# Autodesk Inventor assembly: Ensamblaje2
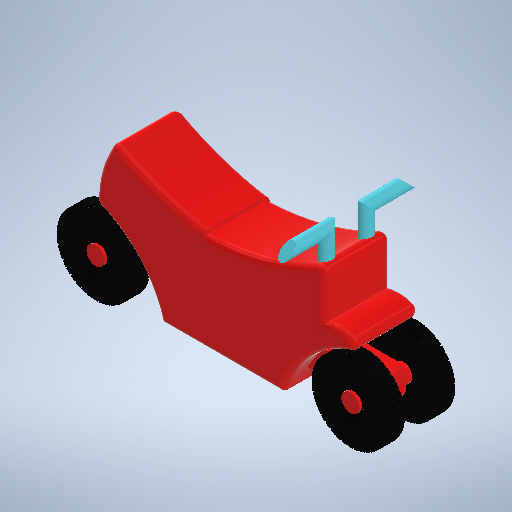
[picture p0: Inventor's stored thumbnail of the model, 512x512]
Saved by Autodesk Inventor 2025.2 (Build 292293000, 293)
## iProperties
Created: 2024-11-29
Part Number: Ensamblaje2
Document SubType Name: Assembly
Designer: usuario
Author: usuario
## Documents named in this file (3)
- C:\Users\usuario\Desktop\APM\ModeladosAPM\Ensamblaje2.iam
- C:\Users\usuario\Desktop\APM\ModeladosAPM\Ensamblajemotocorta.iam
- C:\Users\usuario\Desktop\APM\ModeladosAPM\rueda.ipt
## Components (5 placed, 2 different names)
1. Ensamblajemotocorta:1 [sub-assembly] — Coincidencia:1, Coincidencia:2, Coincidencia:3, Coincidencia:4, Nivelación:1, Nivelación:2, Nivelación:3, Nivelación:4
2. rueda:1 — Coincidencia:1, Nivelación:2
3. rueda:2 — Coincidencia:2, Nivelación:3
4. rueda:3 — Coincidencia:3, Nivelación:1
5. rueda:4 — Coincidencia:4, Nivelación:4
## Relationships (8: Mate 4, Flush 4)
- Coincidencia:1 [Mate]: Ensamblajemotocorta:1 ↔ rueda:1
- Coincidencia:2 [Mate]: Ensamblajemotocorta:1 ↔ rueda:2
- Coincidencia:3 [Mate]: Ensamblajemotocorta:1 ↔ rueda:3
- Coincidencia:4 [Mate]: Ensamblajemotocorta:1 ↔ rueda:4
- Nivelación:1 [Flush]: Ensamblajemotocorta:1 ↔ rueda:3
- Nivelación:2 [Flush]: Ensamblajemotocorta:1 ↔ rueda:1
- Nivelación:3 [Flush]: Ensamblajemotocorta:1 ↔ rueda:2
- Nivelación:4 [Flush]: Ensamblajemotocorta:1 ↔ rueda:4
